# Autodesk Inventor assembly: wheelchair_secure_devices
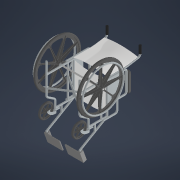
[picture p0: Inventor's stored thumbnail of the model, 180x180]
Saved by Autodesk Inventor 2021 (Build 250183000, 183)
## iProperties
Created: 2021-05-28
Part Number: wheelchair_secure_devices
Document SubType Name: Assembly
Mass: 12088.3 g
Surface Area: 33735.9 cm^2
Volume: 12088.3 cm^3
Density: 1 g/cm^3
## Documents named in this file (3)
- C:\Users\Watchdog\OneDrive - Flinders\Advn Mech Design Shared\6_Development\2_Design\inventor\securing_mechanism\wheelchair_secure_devices.iam
- C:\Users\Watchdog\OneDrive - Flinders\Advn Mech Design Shared\6_Development\2_Design\inventor\vehicle_wheelchair\wheelchair\wheelchair.ipt
- C:\Users\Watchdog\OneDrive - Flinders\Advn Mech Design Shared\6_Development\2_Design\inventor\securing_mechanism\axle_example.ipt
## Components (2 placed, 2 different names)
1. wheelchair:1 — Mate:1, Flush:1
2. axle_example:1 — Mate:1, Flush:2
## Relationships (3: Flush 2, Mate 1)
- Mate:1: wheelchair:1 ↔ axle_example:1
- Flush:1 (220 mm): wheelchair:1
- Flush:2: axle_example:1
